# Autodesk Inventor assembly: framev2
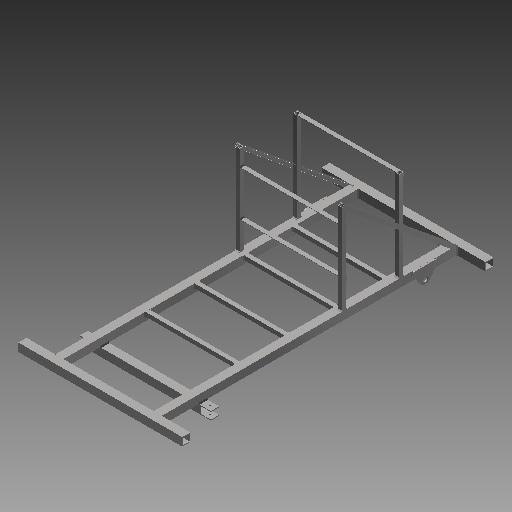
[picture p0: Inventor's stored thumbnail of the model, 512x512]
Saved by Autodesk Inventor 2018 (Build 220112000, 112)
## iProperties
Created: 2018-08-05
Part Number: framev2
Document SubType Name: Weldment
Designer: Cole Tucker
Weld Material: Steel, Mild
Mass: 60664.2 g
Surface Area: 36658.1 cm^2
Volume: 7727.93 cm^3
Density: 7.85 g/cm^3
Author: Cole Tucker
## Documents named in this file (14)
- C:\Users\Cole Tucker\Documents\Github\2018-Personal-Robot\CAD\chassis\Inventor\framev2.iam
- C:\Users\Cole Tucker\Documents\Github\2018-Personal-Robot\CAD\chassis\Inventor\72in2.0Sq.ipt
- C:\Users\Cole Tucker\Documents\Github\2018-Personal-Robot\CAD\chassis\Inventor\22inSqTube.ipt
- C:\Users\Cole Tucker\Documents\Github\2018-Personal-Robot\CAD\chassis\Inventor\32in2.0Sq.ipt
- C:\Users\Cole Tucker\Documents\Github\2018-Personal-Robot\CAD\chassis\Inventor\40in2.0Sq.ipt
- C:\Users\Cole Tucker\Documents\Github\2018-Personal-Robot\CAD\chassis\Inventor\bearingplaterear.ipt
- C:\Users\Cole Tucker\Documents\Github\2018-Personal-Robot\CAD\chassis\Inventor\24in1.0Lch.ipt
- C:\Users\Cole Tucker\Documents\Github\2018-Personal-Robot\CAD\chassis\Inventor\36in1.0Lch.ipt
- C:\Users\Cole Tucker\Documents\Github\2018-Personal-Robot\CAD\chassis\Inventor\framev2\AIP\FEA\clfl0uq3k.fins
- C:\Users\Cole Tucker\Documents\Github\2018-Personal-Robot\CAD\chassis\Inventor\framev2\AIP\FEA\clfl0uq4g.fsat
- C:\Users\Cole Tucker\Documents\Github\2018-Personal-Robot\CAD\chassis\Inventor\framev2\AIP\FEA\clfl0uq4g.ftes
- C:\Users\Cole Tucker\Documents\Github\2018-Personal-Robot\CAD\chassis\Inventor\framev2\AIP\FEA\clfl0uq4g.fwiz
- C:\Users\Cole Tucker\Documents\Github\2018-Personal-Robot\CAD\chassis\Inventor\framev2\AIP\FEA\clfl0uq9s.fmsh
- C:\Users\Cole Tucker\Documents\Github\2018-Personal-Robot\CAD\chassis\Inventor\framev2\AIP\FEA\clfl0uqao.fres
## Components (20 placed, 7 different names)
1. 72in2.0Sq:1 — Mate:1, Mate:2, Mate:3, Mate:4, Flush:1, Flush:2, Flush:3, Flush:4, Flush:5, Flush:6, Flush:7, Flush:8, Flush:9, Flush:10, Mate:6, Flush:11, Mate:8, Flush:16, Mate:11, Flush:18, Mate:15, Mate:16, Flush:21, Flush:22
2. 72in2.0Sq:2 — Mate:5, Flush:5, Flush:6, Flush:12, Mate:7, Flush:13, Flush:14, Mate:9, Flush:17, Mate:13, Mate:14, Flush:19, Flush:20
3. 22inSqTube:1 — Mate:1, Flush:1, Mate:5, Flush:7
4. 22inSqTube:2 — Mate:2, Flush:2, Flush:8
5. 22inSqTube:3 — Mate:3, Flush:3, Flush:9
6. 22inSqTube:4 — Mate:4, Flush:4, Flush:10
7. 32in2.0Sq:1 — Mate:8, Flush:15, Flush:16
8. 40in2.0Sq:1 — Mate:6, Flush:11, Flush:12, Flush:15
9. 40in2.0Sq:2 — Mate:7, Flush:13, Flush:14, Mate:10, Mate:12, Flush:23, Flush:24, Flush:25, Flush:26, Mate:24, Mate:28
10. bearingplaterear:1 — Mate:9, Mate:10, Flush:17
11. bearingplaterear:2 — Mate:11, Mate:12, Flush:18
12. 22inSqTube:5 — Mate:14, Flush:20, Flush:24
13. 22inSqTube:6 — Mate:16, Flush:22, Flush:23, Mate:21, Mate:22, Flush:29, Mate:25
14. 22inSqTube:7 — Mate:15, Flush:21, Flush:25, Mate:26, Mate:30
15. 22inSqTube:8 — Mate:13, Flush:19, Flush:26, Mate:17, Mate:18, Mate:19, Mate:20, Flush:27, Mate:27, Mate:29, Mate:31
16. 24in1.0Lch:2 — Mate:18, Mate:19, Flush:28
17. 24in1.0Lch:3 — Mate:17, Mate:20, Flush:27, Flush:28
18. 24in1.0Lch:4 — Mate:21, Mate:22, Flush:29
19. 36in1.0Lch:1 — Mate:27, Mate:28, Mate:29, Mate:31
20. 36in1.0Lch:2 — Mate:24, Mate:25, Mate:26, Mate:30
## Relationships (59: Mate 30, Flush 29)
- Mate:1: 72in2.0Sq:1 ↔ 22inSqTube:1
- Mate:2: 72in2.0Sq:1 ↔ 22inSqTube:2
- Mate:3: 72in2.0Sq:1 ↔ 22inSqTube:3
- Mate:4: 72in2.0Sq:1 ↔ 22inSqTube:4
- Flush:1: 72in2.0Sq:1 ↔ 22inSqTube:1
- Flush:2: 72in2.0Sq:1 ↔ 22inSqTube:2
- Flush:3: 72in2.0Sq:1 ↔ 22inSqTube:3
- Flush:4: 72in2.0Sq:1 ↔ 22inSqTube:4
- Mate:5: 72in2.0Sq:2 ↔ 22inSqTube:1
- Flush:5: 72in2.0Sq:1 ↔ 72in2.0Sq:2
- Flush:6: 72in2.0Sq:1 ↔ 72in2.0Sq:2
- Flush:7 (508 mm): 72in2.0Sq:1 ↔ 22inSqTube:1
- Flush:8 (812.8 mm): 72in2.0Sq:1 ↔ 22inSqTube:2
- Flush:9 (1117.6 mm): 72in2.0Sq:1 ↔ 22inSqTube:3
- Flush:10 (1422.4 mm): 72in2.0Sq:1 ↔ 22inSqTube:4
- Mate:6: 72in2.0Sq:1 ↔ 40in2.0Sq:1
- Flush:11: 72in2.0Sq:1 ↔ 40in2.0Sq:1
- Flush:12 (-177.8 mm): 72in2.0Sq:2 ↔ 40in2.0Sq:1
- Mate:7: 72in2.0Sq:2 ↔ 40in2.0Sq:2
- Flush:13: 72in2.0Sq:2 ↔ 40in2.0Sq:2
- Flush:14 (-177.8 mm): 72in2.0Sq:2 ↔ 40in2.0Sq:2
- Mate:8: 72in2.0Sq:1 ↔ 32in2.0Sq:1
- Flush:15 (279.4 mm): 32in2.0Sq:1 ↔ 40in2.0Sq:1
- Flush:16 (-76.2 mm): 72in2.0Sq:1 ↔ 32in2.0Sq:1
- Mate:9: 72in2.0Sq:2 ↔ bearingplaterear:1
- Mate:10 (203.2 mm): 40in2.0Sq:2 ↔ bearingplaterear:1
- Flush:17: 72in2.0Sq:2 ↔ bearingplaterear:1
- Mate:11: 72in2.0Sq:1 ↔ bearingplaterear:2
- Mate:12 (203.2 mm): 40in2.0Sq:2 ↔ bearingplaterear:2
- Flush:18: 72in2.0Sq:1 ↔ bearingplaterear:2
- Mate:13: 72in2.0Sq:2 ↔ 22inSqTube:8
- Mate:14: 72in2.0Sq:2 ↔ 22inSqTube:5
- Mate:15: 72in2.0Sq:1 ↔ 22inSqTube:7
- Mate:16: 72in2.0Sq:1 ↔ 22inSqTube:6
- Flush:19: 72in2.0Sq:2 ↔ 22inSqTube:8
- Flush:20: 72in2.0Sq:2 ↔ 22inSqTube:5
- Flush:21: 72in2.0Sq:1 ↔ 22inSqTube:7
- Flush:22: 72in2.0Sq:1 ↔ 22inSqTube:6
- Flush:23 (-355.6 mm): 40in2.0Sq:2 ↔ 22inSqTube:6
- Flush:24 (-355.6 mm): 40in2.0Sq:2 ↔ 22inSqTube:5
- Flush:25 (711.2 mm): 40in2.0Sq:2 ↔ 22inSqTube:7
- Flush:26 (-711.2 mm): 40in2.0Sq:2 ↔ 22inSqTube:8
- Mate:17: 22inSqTube:8 ↔ 24in1.0Lch:3
- Mate:18: 22inSqTube:8 ↔ 24in1.0Lch:2
- Mate:19: 22inSqTube:8 ↔ 24in1.0Lch:2
- Mate:20: 22inSqTube:8 ↔ 24in1.0Lch:3
- Flush:27 (101.6 mm): 22inSqTube:8 ↔ 24in1.0Lch:3
- Flush:28 (279.4 mm): 24in1.0Lch:2 ↔ 24in1.0Lch:3
- Mate:21: 22inSqTube:6 ↔ 24in1.0Lch:4
- Mate:22: 22inSqTube:6 ↔ 24in1.0Lch:4
- Flush:29: 22inSqTube:6 ↔ 24in1.0Lch:4
- Mate:24: 40in2.0Sq:2 ↔ 36in1.0Lch:2
- Mate:25: 22inSqTube:6 ↔ 36in1.0Lch:2
- Mate:26: 22inSqTube:7 ↔ 36in1.0Lch:2
- Mate:27: 22inSqTube:8 ↔ 36in1.0Lch:1
- Mate:28: 40in2.0Sq:2 ↔ 36in1.0Lch:1
- Mate:29: 22inSqTube:8 ↔ 36in1.0Lch:1
- Mate:30: 22inSqTube:7 ↔ 36in1.0Lch:2
- Mate:31: 22inSqTube:8 ↔ 36in1.0Lch:1
## Named parameters: sa_0 = 1.50795e-10, sa_1 = -22241.1, sa_2 = 1.10538e-09, sa_3 = 8.85196e-11, sa_4 = -22241.1, sa_5 = 1.10538e-09
note: some values were not read from the file. Shown as the stored number, unit unknown: "sa_0", "sa_1", "sa_2", "sa_3", "sa_4", "sa_5".
